# Autodesk Inventor assembly: Supershifter Long Hex Output Shaft
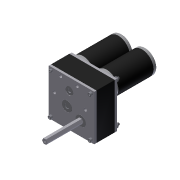
[picture p0: Inventor's stored thumbnail of the model, 180x180]
Saved by Autodesk Inventor 2011 (Build 150239000, 239)
## iProperties
Created: 2012-06-03
Part Number: Supershifter Long Hex Output Shaft
Document SubType Name: Assembly
Designer: Nemo
Author: Nemo
## Documents named in this file (15)
- H:\Nemo\Documents\Robotics\COTS Parts\Gearboxes\Supershifter Long Hex Output Shaft - Left.iam
- H:\Nemo\Documents\Robotics\COTS Parts\Gearboxes\Housings\Supershifter Motor Plate.ipt
- H:\Nemo\Documents\Robotics\COTS Parts\Gearboxes\Shafts\Supershifter Cluster Shaft subassembly.iam
- H:\Nemo\Documents\Robotics\COTS Parts\Gearboxes\Shafts\Supershifter Hex Shaft Standard subassembly.iam
- H:\Nemo\Documents\Robotics\COTS Parts\Gearboxes\Shafts\Supershifter Long Hex Wheel Shaft subassembly.iam
- H:\Nemo\Documents\Robotics\COTS Parts\Gearboxes\Housings\Supershifter Shaft Plate.ipt
- H:\Nemo\Documents\Robotics\COTS Parts\Gearboxes\Shifters\Shifter Cylinder Subassembly.iam
- H:\Nemo\Documents\Robotics\COTS Parts\Fasteners\10-32 locknut.ipt
- H:\Nemo\Documents\Robotics\COTS Parts\Motors\CIM motor 12T for shifters.iam
- H:\Nemo\Documents\Robotics\COTS Parts\Fasteners\14-20 SHCS x3000.ipt
- H:\Nemo\Documents\Robotics\COTS Parts\Fasteners\14-20 locknut.ipt
- H:\Nemo\Documents\Robotics\COTS Parts\Fasteners\10-32 SHCS x2500.ipt
- H:\Nemo\Documents\Robotics\COTS Parts\Fasteners\14-20 captive nut.ipt
- H:\Nemo\Documents\Robotics\COTS Parts\Gearboxes\Housings\Supershifter Enclosure.ipt
- H:\Nemo\Documents\Robotics\COTS Parts\Fasteners\10-32 SHCS x750.ipt
## Components (23 placed, 14 different names)
1. Supershifter Motor Plate:1 — Insert:1, Insert:2, Insert:3, Mate:1, Mate:2, Mate:3, Insert:4, Mate:4, Insert:5, Insert:6, Insert:7, Mate:5, Insert:8, Mate:6, Insert:13, Insert:14, Insert:15, Mate:7, Flush:1, Mate:8, Flush:2, Flush:3, Insert:17, Insert:18, Insert:19, Insert:20
2. Supershifter Cluster Shaft subassembly:1 [sub-assembly] — Insert:3
3. Supershifter Hex Shaft Standard subassembly:1 [sub-assembly] — Insert:2
4. Supershifter Long Hex Wheel Shaft subassembly:1 [sub-assembly] — Insert:1
5. Supershifter Shaft Plate:1 — Mate:1, Mate:2, Mate:3, Insert:9, Insert:11, Insert:12, Insert:21
6. Shifter Cylinder Subassembly:1 [sub-assembly] — Insert:4, Mate:4
7. 10-32 locknut:1 — Insert:5
8. 10-32 locknut:2 — Insert:6
9. CIM motor 12T for shifters:2 [sub-assembly] — Insert:7, Mate:5
10. CIM motor 12T for shifters:1 [sub-assembly] — Insert:8, Mate:6
11. 14-20 SHCS x3000:1 — Insert:9
12. 14-20 SHCS x3000:3 — Insert:11
13. 14-20 SHCS x3000:4 — Insert:12
14. 14-20 locknut:2 — Insert:15
15. 14-20 locknut:3 — Insert:14
16. 14-20 locknut:4 — Insert:13
17. 10-32 SHCS x2500:1 — Insert:21
18. 14-20 captive nut:1 — Mate:7, Flush:1
19. Supershifter Enclosure:1 — Mate:8, Flush:2, Flush:3
20. 10-32 SHCS x750:1 — Insert:17
21. 10-32 SHCS x750:2 — Insert:18
22. 10-32 SHCS x750:3 — Insert:19
23. 10-32 SHCS x750:4 — Insert:20
## Relationships (30: Insert 19, Mate 8, Flush 3)
- Insert:1: Supershifter Motor Plate:1 ↔ Supershifter Long Hex Wheel Shaft subassembly:1
- Insert:2: Supershifter Motor Plate:1 ↔ Supershifter Hex Shaft Standard subassembly:1
- Insert:3: Supershifter Motor Plate:1 ↔ Supershifter Cluster Shaft subassembly:1
- Mate:1: Supershifter Motor Plate:1 ↔ Supershifter Shaft Plate:1
- Mate:2 (50.8 mm): Supershifter Motor Plate:1 ↔ Supershifter Shaft Plate:1
- Mate:3: Supershifter Motor Plate:1 ↔ Supershifter Shaft Plate:1
- Insert:4: Supershifter Motor Plate:1 ↔ Shifter Cylinder Subassembly:1
- Mate:4: Supershifter Motor Plate:1 ↔ Shifter Cylinder Subassembly:1
- Insert:5: Supershifter Motor Plate:1 ↔ 10-32 locknut:1
- Insert:6: Supershifter Motor Plate:1 ↔ 10-32 locknut:2
- Insert:7: Supershifter Motor Plate:1 ↔ CIM motor 12T for shifters:2
- Mate:5: Supershifter Motor Plate:1 ↔ CIM motor 12T for shifters:2
- Insert:8: Supershifter Motor Plate:1 ↔ CIM motor 12T for shifters:1
- Mate:6: Supershifter Motor Plate:1 ↔ CIM motor 12T for shifters:1
- Insert:9: Supershifter Shaft Plate:1 ↔ 14-20 SHCS x3000:1
- Insert:11: Supershifter Shaft Plate:1 ↔ 14-20 SHCS x3000:3
- Insert:12: Supershifter Shaft Plate:1 ↔ 14-20 SHCS x3000:4
- Insert:13: Supershifter Motor Plate:1 ↔ 14-20 locknut:4
- Insert:14: Supershifter Motor Plate:1 ↔ 14-20 locknut:3
- Insert:15: Supershifter Motor Plate:1 ↔ 14-20 locknut:2
- Mate:7: Supershifter Motor Plate:1 ↔ 14-20 captive nut:1
- Flush:1: Supershifter Motor Plate:1 ↔ 14-20 captive nut:1
- Mate:8: Supershifter Motor Plate:1 ↔ Supershifter Enclosure:1
- Flush:2: Supershifter Motor Plate:1 ↔ Supershifter Enclosure:1
- Flush:3: Supershifter Motor Plate:1 ↔ Supershifter Enclosure:1
- Insert:17: Supershifter Motor Plate:1 ↔ 10-32 SHCS x750:1
- Insert:18: Supershifter Motor Plate:1 ↔ 10-32 SHCS x750:2
- Insert:19: Supershifter Motor Plate:1 ↔ 10-32 SHCS x750:3
- Insert:20: Supershifter Motor Plate:1 ↔ 10-32 SHCS x750:4
- Insert:21: Supershifter Shaft Plate:1 ↔ 10-32 SHCS x2500:1
